# Autodesk Inventor assembly: frame
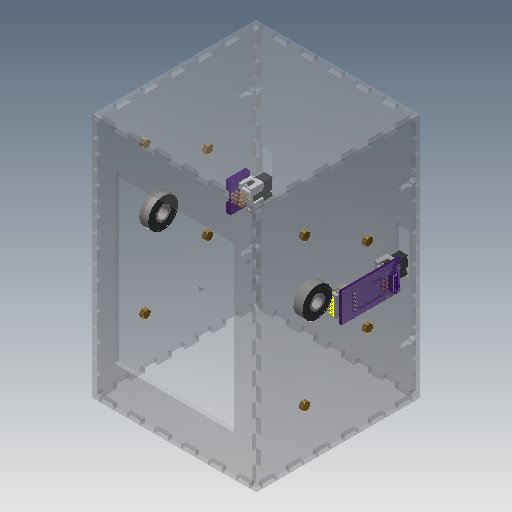
[picture p0: Inventor's stored thumbnail of the model, 512x512]
Saved by Autodesk Inventor 2018 (Build 220112000, 112)
## iProperties
Created: 2015-10-05
Part Number: frame
Document SubType Name: Assembly
Designer: Sawaiz
Author: Sawaiz
## Documents named in this file (6)
- C:\Users\sawaiz\OneDrive\projects\splitFlapDisplay\frame\frame.iam
- C:\Users\sawaiz\OneDrive\projects\splitFlapDisplay\frame\front.ipt
- C:\Users\sawaiz\OneDrive\projects\splitFlapDisplay\frame\back.ipt
- C:\Users\sawaiz\OneDrive\projects\splitFlapDisplay\frame\topBottomPanel.ipt
- C:\Users\sawaiz\OneDrive\projects\splitFlapDisplay\frame\leftSide.iam
- C:\Users\sawaiz\OneDrive\projects\splitFlapDisplay\frame\rightSide.iam
## Components (6 placed, 5 different names)
1. front:1 — Flush:1, Flush:2, Flush:3, Flush:4, Mate:1, Mate:2, Flush:7, Flush:9, Flush:10, Flush:12
2. topBottomPanel:1 — Flush:9, Flush:10, Flush:11
3. topBottomPanel:2 — Flush:7, Flush:8, Flush:12
4. leftSide:1 [sub-assembly] — Flush:2, Flush:4, Mate:1
5. rightSide:1 [sub-assembly] — Flush:1, Flush:3, Flush:5, Flush:6, Mate:2, Flush:8, Flush:11, Flush:13
6. back:1 — Flush:5, Flush:6, Flush:13
## Relationships (15: Flush 13, Mate 2)
- Flush:1: front:1 ↔ rightSide:1
- Flush:2: front:1 ↔ leftSide:1
- Flush:3: front:1 ↔ rightSide:1
- Flush:4: front:1 ↔ leftSide:1
- Flush:5: rightSide:1 ↔ back:1
- Flush:6: rightSide:1 ↔ back:1
- Mate:1: front:1 ↔ leftSide:1
- Mate:2: front:1 ↔ rightSide:1
- Flush:7: front:1 ↔ topBottomPanel:2
- Flush:8: topBottomPanel:2 ↔ rightSide:1
- Flush:9: front:1 ↔ topBottomPanel:1
- Flush:10: front:1 ↔ topBottomPanel:1
- Flush:11: topBottomPanel:1 ↔ rightSide:1
- Flush:12: front:1 ↔ topBottomPanel:2
- Flush:13: rightSide:1 ↔ back:1
